# Autodesk Inventor assembly: FrameAssemblyTest
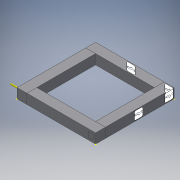
[picture p0: Inventor's stored thumbnail of the model, 180x180]
Saved by Autodesk Inventor 2017 (Build 210142000, 142)
## iProperties
Created: 2018-03-23
Part Number: FrameAssemblyTest
Document SubType Name: Assembly
Designer: User
Mass: 458.838 g
Surface Area: 864.514 cm^2
Volume: 458.838 cm^3
Density: 1 g/cm^3
Author: User
## Documents named in this file (8)
- C:\Robotics\CAD\2018-19_CAD\Offseason\FrameAssemblyTest.iam
- C:\Robotics\CAD\2018-19_CAD\Offseason\FrameAnalysisPart.ipt
- C:\Robotics\CAD\2018-19_CAD\Offseason\FrameAssemblyTest\AIP\FEA\cgkezvatc.fins
- C:\Robotics\CAD\2018-19_CAD\Offseason\FrameAssemblyTest\AIP\FEA\cgkezvatc.fsat
- C:\Robotics\CAD\2018-19_CAD\Offseason\FrameAssemblyTest\AIP\FEA\cgkezvatc.ftes
- C:\Robotics\CAD\2018-19_CAD\Offseason\FrameAssemblyTest\AIP\FEA\cgkezvatc.fwiz
- C:\Robotics\CAD\2018-19_CAD\Offseason\FrameAssemblyTest\AIP\FEA\cgkezvaw0.fmsh
- C:\Robotics\CAD\2018-19_CAD\Offseason\FrameAssemblyTest\AIP\FEA\cgkezvaw1.fres
## Components (4 placed, 1 different names)
1. FrameAnalysisPart:1 — Flush:3, Mate:3, Flush:6
2. FrameAnalysisPart:2 — Flush:1, Mate:1, Flush:2, Flush:3, Flush:4
3. FrameAnalysisPart:3 — Flush:4, Mate:2, Flush:5, Mate:3, Flush:6
4. FrameAnalysisPart:4 — Flush:1, Mate:1, Flush:2, Mate:2, Flush:5
## Relationships (9: Flush 6, Mate 3)
- Flush:1: FrameAnalysisPart:2 ↔ FrameAnalysisPart:4
- Mate:1: FrameAnalysisPart:2 ↔ FrameAnalysisPart:4
- Flush:2: FrameAnalysisPart:2 ↔ FrameAnalysisPart:4
- Flush:3: FrameAnalysisPart:1 ↔ FrameAnalysisPart:2
- Flush:4: FrameAnalysisPart:2 ↔ FrameAnalysisPart:3
- Mate:2: FrameAnalysisPart:3 ↔ FrameAnalysisPart:4
- Flush:5: FrameAnalysisPart:3 ↔ FrameAnalysisPart:4
- Mate:3: FrameAnalysisPart:1 ↔ FrameAnalysisPart:3
- Flush:6: FrameAnalysisPart:1 ↔ FrameAnalysisPart:3
## Named parameters: sa_0 = 4448.22, sa_1 = 0, sa_2 = 0
note: some values were not read from the file. Shown as the stored number, unit unknown: "sa_0", "sa_1", "sa_2".
